# Autodesk Inventor assembly: item_0042502_winkelsatz_5_20x20_details_3_Grundplatte
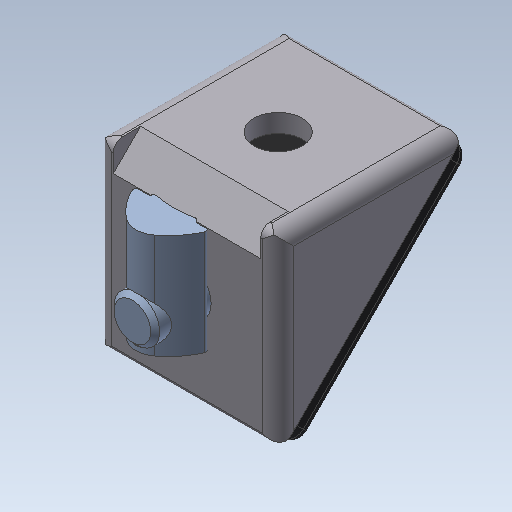
[picture p0: Inventor's stored thumbnail of the model, 512x512]
Saved by Autodesk Inventor 2021 (Build 250183000, 183)
## iProperties
Company: TraceParts S.A.
Created: 2021-02-17
Part Number: item_0042502_winkelsatz_5_20x20_details_3_Grundplatte
Checked By: TraceParts S.A.
Catalog Web Link: www.traceparts.com
Document SubType Name: Assembly
Designer: TraceParts
REFERENCE: 0.0.425.02
SUPPLIER: item Industrietechnik GmbH
DESIGN: Winkelsatz 5 20x20
SELECTION: 0.0.425.02
TraceParts.PartVersion: 1.0.1
TraceParts.PartStatus: Published
TraceParts.PartNumber: 30-12112020-080175
TraceParts.PartLanguage: de
TraceParts.InstanceId: 30-12112020-080175775LNV7JRFOC89W6054LU0LGS
TraceParts.PartTitle: Winkelsatz 5 20x20
TRACEPARTS: TRACEPARTS
TraceParts.ClassPath: ITEM:30-12112020-080175
Author: TraceParts
## Documents named in this file (5)
- C:\Users\Sebastian Seewald\Documents\Inventor\Konstruktion_Studium\Lernfabrik\102_Rahmen_Modul\202.001.01_ZB_ITEM_Winkelsatz_5_20x20.iam
- C:\Users\Sebastian Seewald\Documents\Inventor\Konstruktion_Studium\Lernfabrik\102_Rahmen_Modul\502.012.01_ITEM_Stahlwinkel_5_20x20.ipt
- C:\Users\Sebastian Seewald\Documents\Inventor\Konstruktion_Studium\Lernfabrik\102_Rahmen_Modul\502.015.01_ITEM_Abdeckung_5_20x20.ipt
- C:\Users\Sebastian Seewald\Documents\Inventor\Konstruktion_Studium\Lernfabrik\102_Rahmen_Modul\502.013.01_ITEM_Winkelschraube_5_20x20.ipt
- C:\Users\Sebastian Seewald\Documents\Inventor\Konstruktion_Studium\Lernfabrik\102_Rahmen_Modul\502.014.01_ITEM_Stein_5_20x20.ipt
## Components (4 placed, 4 different names)
1. 502.012.01_ITEM_Stahlwinkel_5_20x20:1 — Passend:3, Passend:4, Passend:5, Passend:6, Passend:7, Passend:8, Winkel:1
2. 502.015.01_ITEM_Abdeckung_5_20x20:1 — Passend:5, Passend:6, Passend:7
3. 502.013.01_ITEM_Winkelschraube_5_20x20:1 — Passend:3, Passend:4, Passend:9
4. 502.014.01_ITEM_Stein_5_20x20:1 — Passend:8, Passend:9, Winkel:1
## Relationships (8: Mate 7, Angle 1)
- Passend:3 [Mate]: 502.012.01_ITEM_Stahlwinkel_5_20x20:1 ↔ 502.013.01_ITEM_Winkelschraube_5_20x20:1
- Passend:4 [Mate]: 502.012.01_ITEM_Stahlwinkel_5_20x20:1 ↔ 502.013.01_ITEM_Winkelschraube_5_20x20:1
- Passend:5 [Mate]: 502.012.01_ITEM_Stahlwinkel_5_20x20:1 ↔ 502.015.01_ITEM_Abdeckung_5_20x20:1
- Passend:6 [Mate]: 502.012.01_ITEM_Stahlwinkel_5_20x20:1 ↔ 502.015.01_ITEM_Abdeckung_5_20x20:1
- Passend:7 [Mate]: 502.012.01_ITEM_Stahlwinkel_5_20x20:1 ↔ 502.015.01_ITEM_Abdeckung_5_20x20:1
- Passend:8 [Mate] (1.6 mm): 502.012.01_ITEM_Stahlwinkel_5_20x20:1 ↔ 502.014.01_ITEM_Stein_5_20x20:1
- Passend:9 [Mate]: 502.013.01_ITEM_Winkelschraube_5_20x20:1 ↔ 502.014.01_ITEM_Stein_5_20x20:1
- Winkel:1 [Angle] (180 deg): 502.012.01_ITEM_Stahlwinkel_5_20x20:1 ↔ 502.014.01_ITEM_Stein_5_20x20:1
